# Autodesk Inventor assembly: ZlozenieDwochSuperCzesci
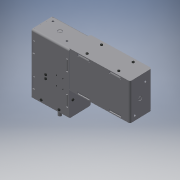
[picture p0: Inventor's stored thumbnail of the model, 180x180]
Saved by Autodesk Inventor 2019 (Build 230136000, 136)
## iProperties
Created: 2020-08-29
Part Number: ZlozenieDwochSuperCzesci
Document SubType Name: Assembly
Designer: estee
Author: estee
## Documents named in this file (3)
- C:\Users\estee\OneDrive\Pulpit\estere\1\MUM\nowygit\Mechanika\Moduł obrotu DEK Bartek\odBartka\ZlozenieDwochSuperCzesci.iam
- C:\Users\estee\OneDrive\Pulpit\estere\1\MUM\nowygit\Mechanika\Moduł obrotu DEK Bartek\odBartka\Moduł1.iam
- C:\Users\estee\OneDrive\Pulpit\estere\1\MUM\nowygit\Mechanika\Moduł obrotu DEK Bartek\odBartka\Moduł3.iam
## Components (2 placed, 2 different names)
1. Moduł1:1 [sub-assembly] — Mate:1, Angle:1, Flush:1
2. Moduł3:1 [sub-assembly] — Mate:1, Angle:1, Flush:1
## Relationships (3: Mate 1, Angle 1, Flush 1)
- Mate:1: Moduł1:1 ↔ Moduł3:1
- Angle:1 (0 deg): Moduł1:1 ↔ Moduł3:1
- Flush:1: Moduł1:1 ↔ Moduł3:1
